# Autodesk Inventor assembly: ASY GBK bottom 0010
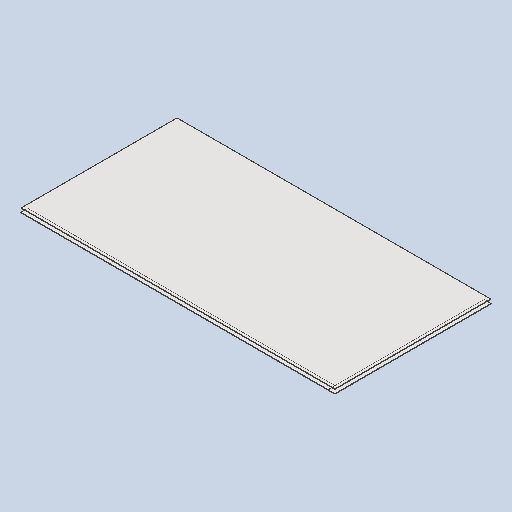
[picture p0: Inventor's stored thumbnail of the model, 512x512]
Saved by Autodesk Inventor 2026.2 (Build 302298000, 298)
## iProperties
Created: 2026-07-09
Part Number: ASY GBK bottom 0010
Document SubType Name: Assembly
Designer: admin
Stock Number: 0010
Author: admin
## Documents named in this file (4)
- C:\Users\admin\Documents\Inventor\GBK-Gubkinskiy\ASY GBK bottom 0010.iam
- C:\Users\admin\Documents\Inventor\GBK-Gubkinskiy\Пол\GBK bottom 0135.ipt
- C:\Users\admin\Documents\Inventor\GBK-Gubkinskiy\Пол\GBK bottom 0134.ipt
- C:\Users\admin\Documents\Inventor\GBK-Gubkinskiy\Пол\GBK bottom 0125.ipt
## Components (3 placed, 3 different names)
1. GBK bottom 0135:1
2. GBK bottom 0134:1
3. GBK bottom 0125:1
## Relationships (4: Mate 3, WeldJoint 1)
- [WeldJoint]: GBK bottom 0135:1 ↔ GBK bottom 0134:1
- [Mate] (-30 mm): GBK bottom 0134:1 ↔ GBK bottom 0125:1
- [Mate] (-30 mm): GBK bottom 0135:1 ↔ GBK bottom 0125:1
- [Mate]: GBK bottom 0134:1 ↔ GBK bottom 0125:1
